# Autodesk Inventor assembly: 000.005 -  Манипулятор
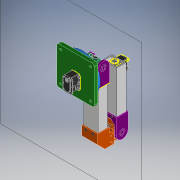
[picture p0: Inventor's stored thumbnail of the model, 180x180]
Saved by Autodesk Inventor 2022 (Build 260153000, 153)
## iProperties
Created: 2022-11-17
Part Number: 000.005 -  Манипулятор
Document SubType Name: Assembly
Designer: Petrov Ivan
Author: Petrov Ivan
## Documents named in this file (7)
- D:\IVAN\Ivan_desktop\Kvantorium\Projects\YouBotRobot\design\000.005 -  Манипулятор.iam
- D:\IVAN\Ivan_desktop\Kvantorium\Projects\YouBotRobot\design\000.005.001 - Поворотный стол.iam
- D:\IVAN\Ivan_desktop\Kvantorium\Projects\YouBotRobot\design\000.005.002 - Плечо СБ.iam
- D:\IVAN\Ivan_desktop\Kvantorium\Projects\YouBotRobot\design\000.005.003 - Локоть СБ.iam
- C:\Users\Petrov Ivan\Documents\Inventor\Content Center Files\R2022\ru-RU\ISO 4762(1)\DIN EN ISO 4762 - M4 x 16.ipt
- D:\IVAN\Ivan_desktop\Kvantorium\Projects\YouBotRobot\design\standart_components\dynamixels\mx-28\MX-28.iam
- D:\IVAN\Ivan_desktop\Kvantorium\Projects\YouBotRobot\design\standart_components\dynamixels\mx-64\MX-64T.iam
## Components (9 placed, 6 different names)
1. 000.005.001 - Поворотный стол СБ:1 [sub-assembly] — Совмещение:1, Совмещение:2, Совмещение:3, Угол:1, Угол:2
2. 000.005.002 - Плечо СБ:1 [sub-assembly] — Совмещение:1, Совмещение:2, Совмещение:3, Вставка:1, Вставка:2, Вставка:3, Вставка:4, Угол:1, Совмещение:4, Совмещение:5, Совмещение:6, Угол:2, Угол:3
3. 000.005.003 - Локоть СБ:1 [sub-assembly] — Совмещение:4, Совмещение:5, Совмещение:6, Угол:3, Совмещение:7, Угол:4, Совмещение:9, Угол:5, Заподлицо:1, Угол:6
4. DIN EN ISO 4762 M4 x 16:1 — Вставка:1
5. DIN EN ISO 4762 M4 x 16:2 — Вставка:2
6. DIN EN ISO 4762 M4 x 16:3 — Вставка:3
7. DIN EN ISO 4762 M4 x 16:4 — Вставка:4
8. MX-28:1 [sub-assembly]
9. MX-64T:1 [sub-assembly] — Совмещение:8, Совмещение:10, Заподлицо:1, Угол:6
## Relationships (21: Mate 10, Angle 6, Insert 4, Flush 1)
- Совмещение:1 [Mate]: 000.005.001 - Поворотный стол СБ:1 ↔ 000.005.002 - Плечо СБ:1
- Совмещение:2 [Mate]: 000.005.001 - Поворотный стол СБ:1 ↔ 000.005.002 - Плечо СБ:1
- Совмещение:3 [Mate]: 000.005.001 - Поворотный стол СБ:1 ↔ 000.005.002 - Плечо СБ:1
- Вставка:1 [Insert]: 000.005.002 - Плечо СБ:1 ↔ DIN EN ISO 4762 M4 x 16:1
- Вставка:2 [Insert]: 000.005.002 - Плечо СБ:1 ↔ DIN EN ISO 4762 M4 x 16:2
- Вставка:3 [Insert]: 000.005.002 - Плечо СБ:1 ↔ DIN EN ISO 4762 M4 x 16:3
- Вставка:4 [Insert]: 000.005.002 - Плечо СБ:1 ↔ DIN EN ISO 4762 M4 x 16:4
- Угол:1 [Angle] (180 deg): 000.005.001 - Поворотный стол СБ:1 ↔ 000.005.002 - Плечо СБ:1
- Совмещение:4 [Mate]: 000.005.002 - Плечо СБ:1 ↔ 000.005.003 - Локоть СБ:1
- Совмещение:5 [Mate] (0.25 mm): 000.005.002 - Плечо СБ:1 ↔ 000.005.003 - Локоть СБ:1
- Совмещение:6 [Mate] (0.25 mm): 000.005.002 - Плечо СБ:1 ↔ 000.005.003 - Локоть СБ:1
- Угол:2 [Angle] (0 deg): 000.005.001 - Поворотный стол СБ:1 ↔ 000.005.002 - Плечо СБ:1
- Угол:3 [Angle] (0 deg): 000.005.002 - Плечо СБ:1 ↔ 000.005.003 - Локоть СБ:1
- Совмещение:7 [Mate]: 000.005.003 - Локоть СБ:1
- Угол:4 [Angle] (0 deg): 000.005.003 - Локоть СБ:1
- Совмещение:8 [Mate]: MX-64T:1
- Совмещение:9 [Mate]: 000.005.003 - Локоть СБ:1
- Угол:5 [Angle] (0 deg): 000.005.003 - Локоть СБ:1
- Совмещение:10 [Mate]: MX-64T:1
- Заподлицо:1 [Flush]: 000.005.003 - Локоть СБ:1 ↔ MX-64T:1
- Угол:6 [Angle] (0 deg): 000.005.003 - Локоть СБ:1 ↔ MX-64T:1
